# Autodesk Inventor assembly: rigt_motor_asembly
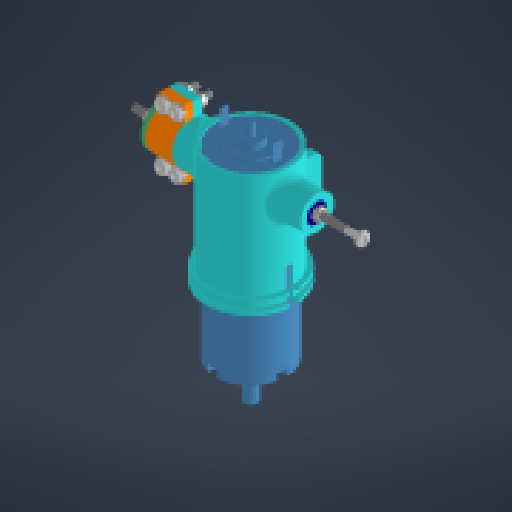
[picture p0: Inventor's stored thumbnail of the model, 512x512]
Saved by Autodesk Inventor 2024 (Build 280153000, 153)
## iProperties
Created: 2023-05-14
Part Number: rigt_motor_asembly
Document SubType Name: Assembly
Designer: user
Mass: 529.807 g
Surface Area: 912.469 cm^2
Volume: 506.199 cm^3
Density: 1.04664 g/cm^3
Author: user
## Documents named in this file (11)
- D:\Docs\Robot\3d\motor_assembly\rigt_motor_asembly.iam
- D:\Docs\Robot\3d\motor_assembly\rigt_motor_asembly\lower_arm.ipt
- D:\Docs\Robot\3d\motor_assembly\bushing_assembly.iam
- D:\Docs\Robot\3d\default_components\motor.ipt
- D:\Docs\Robot\3d\default_components\604zz_bearing.ipt
- C:\Users\user\Documents\Inventor\Content Center Files\R2024\ru-RU\DIN 934\DIN 934 - M4 x 0,7.ipt
- C:\Users\user\Documents\Inventor\Content Center Files\R2024\ru-RU\DIN 7985 (H)\DIN 7985 (H) - M4x30-H.ipt
- D:\Docs\Robot\3d\motor_assembly\default_motor_asembly\cup.ipt
- C:\Users\user\Documents\Inventor\Content Center Files\R2024\ru-RU\DIN 125-1  A\DIN 125 - A 4,3.ipt
- C:\Users\user\Documents\Inventor\Content Center Files\R2024\ru-RU\DIN 7985 (H)\DIN 7985 (H) - M4x20-H.ipt
- D:\Docs\Robot\3d_v2\machine_body\wheel_assembly.iam
## Components (24 placed, 10 different names)
1. lower_arm:1 — Совмещение:1, Совмещение:2, Совмещение:3, Совмещение:4, Вставка:5, Вставка:7, Заподлицо:1, Вставка:12, Вставка:13, Вставка:18, Вставка:19, Вставка:20, Вставка:21, Вставка:31
2. bushing_assembly:2 [sub-assembly] — Заподлицо:1, Вставка:31
3. motor:1 — Вставка:5, Вставка:30
4. 604zz_bearing:1 — Вставка:7, Вставка:8, Вставка:11
5. DIN 934 - заменено на DIN EN 24032/28673/28674 M4:1 — Вставка:8
6. DIN 7985 (H) M4x30-H:1 — Вставка:11
7. cup:1 — Вставка:12, Вставка:13, Вставка:14, Вставка:15, Вставка:16, Вставка:17
8. DIN 125-1 A A 4,3:1 — Вставка:14, Вставка:24
9. DIN 125-1 A A 4,3:2 — Вставка:15, Вставка:25
10. DIN 125-1 A A 4,3:3 — Вставка:16, Вставка:22
11. DIN 125-1 A A 4,3:4 — Вставка:17, Вставка:23
12. DIN 125-1 A A 4,3:5 — Вставка:18, Вставка:27
13. DIN 125-1 A A 4,3:6 — Вставка:19, Вставка:26
14. DIN 125-1 A A 4,3:7 — Вставка:20, Вставка:28
15. DIN 125-1 A A 4,3:8 — Вставка:21, Вставка:29
16. DIN 7985 (H) M4x20-H:1 — Вставка:25
17. DIN 7985 (H) M4x20-H:2 — Вставка:24
18. DIN 7985 (H) M4x20-H:3 — Вставка:23
19. DIN 7985 (H) M4x20-H:4 — Вставка:22
20. DIN 934 - заменено на DIN EN 24032/28673/28674 M4:2 — Вставка:26
21. DIN 934 - заменено на DIN EN 24032/28673/28674 M4:3 — Вставка:27
22. DIN 934 - заменено на DIN EN 24032/28673/28674 M4:4 — Вставка:29
23. DIN 934 - заменено на DIN EN 24032/28673/28674 M4:5 — Вставка:28
24. wheel_assembly:1 [sub-assembly] — Вставка:30
## Relationships (29: Insert 24, Mate 4, Flush 1)
- Совмещение:1 [Mate]: lower_arm:1
- Совмещение:2 [Mate]: lower_arm:1
- Совмещение:3 [Mate]: lower_arm:1
- Совмещение:4 [Mate]: lower_arm:1
- Вставка:5 [Insert]: lower_arm:1 ↔ motor:1
- Вставка:7 [Insert]: lower_arm:1 ↔ 604zz_bearing:1
- Вставка:8 [Insert]: 604zz_bearing:1 ↔ DIN 934 - заменено на DIN EN 24032/28673/28674 M4:1
- Вставка:11 [Insert]: 604zz_bearing:1 ↔ DIN 7985 (H) M4x30-H:1
- Заподлицо:1 [Flush]: lower_arm:1 ↔ bushing_assembly:2
- Вставка:12 [Insert]: lower_arm:1 ↔ cup:1
- Вставка:13 [Insert]: lower_arm:1 ↔ cup:1
- Вставка:14 [Insert]: cup:1 ↔ DIN 125-1 A A 4,3:1
- Вставка:15 [Insert]: cup:1 ↔ DIN 125-1 A A 4,3:2
- Вставка:16 [Insert]: cup:1 ↔ DIN 125-1 A A 4,3:3
- Вставка:17 [Insert]: cup:1 ↔ DIN 125-1 A A 4,3:4
- Вставка:18 [Insert]: lower_arm:1 ↔ DIN 125-1 A A 4,3:5
- Вставка:19 [Insert]: lower_arm:1 ↔ DIN 125-1 A A 4,3:6
- Вставка:20 [Insert]: lower_arm:1 ↔ DIN 125-1 A A 4,3:7
- Вставка:21 [Insert]: lower_arm:1 ↔ DIN 125-1 A A 4,3:8
- Вставка:22 [Insert]: DIN 125-1 A A 4,3:3 ↔ DIN 7985 (H) M4x20-H:4
- Вставка:23 [Insert]: DIN 125-1 A A 4,3:4 ↔ DIN 7985 (H) M4x20-H:3
- Вставка:24 [Insert]: DIN 125-1 A A 4,3:1 ↔ DIN 7985 (H) M4x20-H:2
- Вставка:25 [Insert]: DIN 125-1 A A 4,3:2 ↔ DIN 7985 (H) M4x20-H:1
- Вставка:26 [Insert]: DIN 125-1 A A 4,3:6 ↔ DIN 934 - заменено на DIN EN 24032/28673/28674 M4:2
- Вставка:27 [Insert]: DIN 125-1 A A 4,3:5 ↔ DIN 934 - заменено на DIN EN 24032/28673/28674 M4:3
- Вставка:28 [Insert]: DIN 125-1 A A 4,3:7 ↔ DIN 934 - заменено на DIN EN 24032/28673/28674 M4:5
- Вставка:29 [Insert]: DIN 125-1 A A 4,3:8 ↔ DIN 934 - заменено на DIN EN 24032/28673/28674 M4:4
- Вставка:30 [Insert]: motor:1 ↔ wheel_assembly:1
- Вставка:31 [Insert]: lower_arm:1 ↔ bushing_assembly:2
